# Autodesk Inventor assembly: 537247 FNC-20
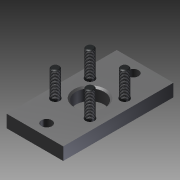
[picture p0: Inventor's stored thumbnail of the model, 180x180]
Saved by Autodesk Inventor 2011 SP1 (Build 150282100, 282)
## iProperties
Created: 2018-05-29
Part Number: 537247 FNC-20
Catalog Web Link: www.cadenas.de
Description: FNC-Flange mounting
Vendor: FESTO
Document SubType Name: Assembly
Designer: psAdmin
Manufacturer: FESTO
Mass: 141 g
Category: PARTsolutions
Company: FESTO
Title: 537247 FNC-20
Author: Cadenas PARTsolutions
Comments: Flange mounting
PSOL_IDENT_0: {$CADENAS_DATA\23d-libs\festo\parts\f\fnc\fnc_asmtab.prj},180 {VTYP=3D},{STYP=ASSTAB},{NB=537247 FNC
PSOL_IDENT_1: -20},{LINA=537247 FNC-20},{NN=FNC},{DATE=02.09.2015 15:05:29},{GEOMDATE=02.09.2015 15:05:29},{VERSIO
PSOL_IDENT_2: N=},{LINEID=110},{LINESUBID=-1},{WBVAR=}  {NB=537247 FNC-20},{LINA=537247 FNC-20},{KT=DUMMY},{TNR=53
PSOL_IDENT_3: 7247},{TYP=FNC-20},{VERS=1},{D1=18.000},{D2=5.800},{D3=10.000},{E=36.000},{F=1.000},{FB=6.600},{MF=8
PSOL_IDENT_4: .000},{R=0.000},{T=3.000},{TF=55.000},{TG1=22.000},{UF=70.000},{CNSMASSEXACT=0.141},{ZZ=0},{DK=20},{
PSOL_IDENT_5: D6912D=5.000},{D6912L=20.000},{PPATH=assemblies/fnc_asmtpl.prj}
NN: FNC
NT: Flange mounting
NB: 537247 FNC-20
NBSYN: $TNR. $TYP.
LINA: 537247 FNC-20
TNR: 537247
TYP: FNC-20
D1: 18.000
D2: 5.800
D3: 10.000
E: 36.000
F: 1.000
FB: 6.600
MF: 8.000
R: 0.000
T: 3.000
TF: 55.000
TG1: 22.000
UF: 70.000
CNSMASSEXACT: 0.141
SUPPLIER: FESTO
ARTICLENO: 537247 FNC-20
BOMINFO: 537247 FNC-20
CREATOR: CADENAS GmbH
## Documents named in this file (3)
- p:\temp\worker_3\2196_1416\cad_40_02018052911532467432116192d056f_000000_00_00_000001\537247 FNC-20.iam
- p:\temp\worker_3\2196_1416\cad_40_02018052911532467432116192d056f_000000_00_00_000001\537247 FNC-20---(F).ipt
- p:\temp\worker_3\2196_1416\cad_40_02018052911532467432116192d056f_000000_00_00_000001\DIN-6912 - M5x20(F).ipt
## Components (5 placed, 2 different names)
1. 537247 FNC-20---(F):1 — FNC_Schraube_1_XY@1 <-> MONTAGE_XY@2, FNC_Schraube_1_Z@1 <-> MONTAGE_Z@2, FNC_Schraube_2_XY@1 <-> MONTAGE_XY@3, FNC_Schraube_2_Z@1 <-> MONTAGE_Z@3, FNC_Schraube_2_YZ@1 <-> MONTAGE_YZ@3, FNC_Schraube_3_XY@1 <-> MONTAGE_XY@4, FNC_Schraube_3_Z@1 <-> MONTAGE_Z@4, FNC_Schraube_3_YZ@1 <-> MONTAGE_YZ@4, FNC_Schraube_4_XY@1 <-> MONTAGE_XY@5, FNC_Schraube_4_Z@1 <-> MONTAGE_Z@5
2. DIN-6912 - M5x20(F):1 — FNC_Schraube_1_XY@1 <-> MONTAGE_XY@2, FNC_Schraube_1_Z@1 <-> MONTAGE_Z@2
3. DIN-6912 - M5x20(F):2 — FNC_Schraube_2_XY@1 <-> MONTAGE_XY@3, FNC_Schraube_2_Z@1 <-> MONTAGE_Z@3, FNC_Schraube_2_YZ@1 <-> MONTAGE_YZ@3
4. DIN-6912 - M5x20(F):3 — FNC_Schraube_3_XY@1 <-> MONTAGE_XY@4, FNC_Schraube_3_Z@1 <-> MONTAGE_Z@4, FNC_Schraube_3_YZ@1 <-> MONTAGE_YZ@4
5. DIN-6912 - M5x20(F):4 — FNC_Schraube_4_XY@1 <-> MONTAGE_XY@5, FNC_Schraube_4_Z@1 <-> MONTAGE_Z@5
## Relationships (10: Flush 4, Mate 4, Angle 2)
- FNC_Schraube_1_XY@1 <-> MONTAGE_XY@2 [Flush]: 537247 FNC-20---(F):1 ↔ DIN-6912 - M5x20(F):1
- FNC_Schraube_1_Z@1 <-> MONTAGE_Z@2 [Mate]: 537247 FNC-20---(F):1 ↔ DIN-6912 - M5x20(F):1
- FNC_Schraube_2_XY@1 <-> MONTAGE_XY@3 [Flush]: 537247 FNC-20---(F):1 ↔ DIN-6912 - M5x20(F):2
- FNC_Schraube_2_Z@1 <-> MONTAGE_Z@3 [Mate]: 537247 FNC-20---(F):1 ↔ DIN-6912 - M5x20(F):2
- FNC_Schraube_2_YZ@1 <-> MONTAGE_YZ@3 [Angle] (0 deg): 537247 FNC-20---(F):1 ↔ DIN-6912 - M5x20(F):2
- FNC_Schraube_3_XY@1 <-> MONTAGE_XY@4 [Flush]: 537247 FNC-20---(F):1 ↔ DIN-6912 - M5x20(F):3
- FNC_Schraube_3_Z@1 <-> MONTAGE_Z@4 [Mate]: 537247 FNC-20---(F):1 ↔ DIN-6912 - M5x20(F):3
- FNC_Schraube_3_YZ@1 <-> MONTAGE_YZ@4 [Angle] (0 deg): 537247 FNC-20---(F):1 ↔ DIN-6912 - M5x20(F):3
- FNC_Schraube_4_XY@1 <-> MONTAGE_XY@5 [Flush]: 537247 FNC-20---(F):1 ↔ DIN-6912 - M5x20(F):4
- FNC_Schraube_4_Z@1 <-> MONTAGE_Z@5 [Mate]: 537247 FNC-20---(F):1 ↔ DIN-6912 - M5x20(F):4
